# Autodesk Inventor assembly: Assembly2
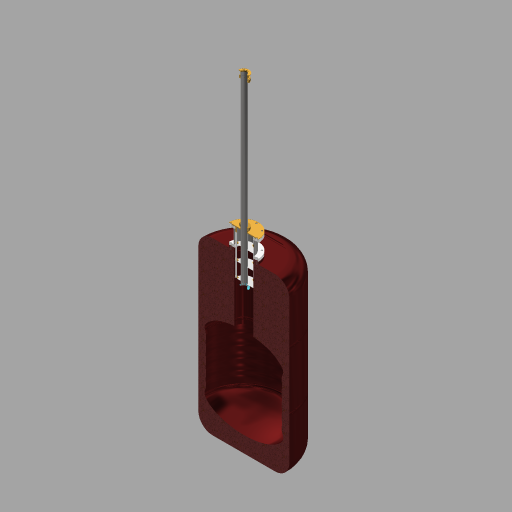
[picture p0: Inventor's stored thumbnail of the model, 512x512]
Saved by Autodesk Inventor 2024 (Build 280153020, 153B)
## iProperties
Created: 2023-10-25
Part Number: Assembly2
Document SubType Name: Assembly
Designer: schanen
Author: schanen
## Documents named in this file (5)
- C:\Users\schanen\Documents\Inventor\LargeTransportDewarInsert2023\Assembly2.iam
- C:\Users\schanen\Documents\Inventor\LargeTransportDewarInsert2023\Collar.iam
- C:\Users\schanen\Documents\Inventor\LargeTransportDewarInsert2023\TransportDewar.ipt
- C:\Users\schanen\Documents\Inventor\LargeTransportDewarInsert2023\SlidingAssembly.iam
- C:\Users\schanen\Documents\Inventor\LargeTransportDewarInsert2023\Insert2.iam
## Components (4 placed, 4 different names)
1. Collar:1 [sub-assembly] — Mate:1, Mate:3, Mate:4, Mate:5
2. TransportDewar:1 — Mate:1, Mate:2, Mate:3, Flush:5, Mate:4
3. Insert2:1 [sub-assembly]
4. SlidingAssembly:1 [sub-assembly]
## Relationships (10: Mate 8, Flush 1, Tangent 1)
- Mate:1: Collar:1 ↔ TransportDewar:1
- Mate:2: TransportDewar:1
- Mate:3: Collar:1 ↔ TransportDewar:1
- Flush:5: TransportDewar:1
- Mate:4: Collar:1 ↔ TransportDewar:1
- Mate:5: Collar:1
- [Mate]: Collar:1 ↔ Insert2:1
- [Tangent]: Collar:1 ↔ Insert2:1
- [Mate]: Collar:1 ↔ Insert2:1
- [Mate]: Insert2:1 ↔ SlidingAssembly:1
